# Autodesk Inventor assembly: rackpinion.ipt
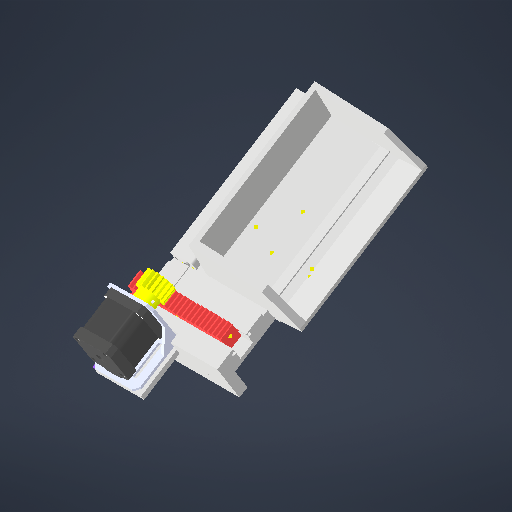
[picture p0: Inventor's stored thumbnail of the model, 512x512]
Saved by Autodesk Inventor 2027 (Build 310192000, 192)
## iProperties
Created: 2026-07-10
Part Number: rackpinion.ipt
Document SubType Name: Assembly
Designer: uchiha
Author: uchiha
## Documents named in this file (8)
- C:\Users\uchiha\Desktop\New folder\designdj\rackpinion.ipt.iam
- C:\Users\uchiha\Desktop\New folder\designdj\offloadbase.ipt
- C:\Users\uchiha\Desktop\New folder\designdj\gearsassembly.iam
- C:\Users\uchiha\Desktop\New folder\designdj\nema17-4-4kgcm-stepper-motor-1.snapshot.1\Nema17 4.4Kgcm Stepper Motor\Nema17 4.4Kgcm Stepper Motor\Nema17 4.4Kgcm Stepper Motor.iam
- C:\Users\uchiha\Desktop\New folder\designdj\Assemblyplates.iam
- C:\Users\uchiha\Documents\Inventor\Content Center Files\R2027\en-US\AS 1110\AS 1110 - M2 x 16.ipt
- C:\Users\uchiha\Documents\Inventor\Content Center Files\R2027\en-US\AS 1112 (2)\AS 1112 - M2  Type 5.ipt
- C:\Users\uchiha\Desktop\New folder\designdj\rockerconnector.ipt
## Components (9 placed, 7 different names)
1. offloadbase:1 — Mate:1, Mate:2, Mate:12, Mate:16, Mate:17
2. gearsassembly:1 [sub-assembly] — Mate:1, Mate:2, Mate:15, Mate:18, Mate:19
3. Nema17 4.4Kgcm Stepper Motor:1 [sub-assembly] — Mate:15
4. Assemblyplates:1 [sub-assembly] — Insert:1, Insert:2, Mate:7, Mate:9, Mate:10, Mate:12, Mate:16, Mate:17
5. AS 1110 - Metric M2 x 16:1 — Insert:1, Mate:5, Mate:10, Mate:13, Mate:14
6. AS 1110 - Metric M2 x 16:2 — Insert:2, Mate:6, Mate:9
7. AS 1112 (2) - Metric M2  Type 5:1 — Mate:5, Mate:13, Mate:14
8. AS 1112 (2) - Metric M2  Type 5:2 — Mate:6, Mate:7
9. rockerconnector:1 — Mate:18, Mate:19
## Relationships (17: Mate 15, Insert 2)
- Mate:1: offloadbase:1 ↔ gearsassembly:1
- Mate:2: offloadbase:1 ↔ gearsassembly:1
- Insert:1: Assemblyplates:1 ↔ AS 1110 - Metric M2 x 16:1
- Insert:2: Assemblyplates:1 ↔ AS 1110 - Metric M2 x 16:2
- Mate:5: AS 1110 - Metric M2 x 16:1 ↔ AS 1112 (2) - Metric M2  Type 5:1
- Mate:6: AS 1110 - Metric M2 x 16:2 ↔ AS 1112 (2) - Metric M2  Type 5:2
- Mate:7: Assemblyplates:1 ↔ AS 1112 (2) - Metric M2  Type 5:2
- Mate:9: Assemblyplates:1 ↔ AS 1110 - Metric M2 x 16:2
- Mate:10: Assemblyplates:1 ↔ AS 1110 - Metric M2 x 16:1
- Mate:12: offloadbase:1 ↔ Assemblyplates:1
- Mate:13: AS 1110 - Metric M2 x 16:1 ↔ AS 1112 (2) - Metric M2  Type 5:1
- Mate:14: AS 1110 - Metric M2 x 16:1 ↔ AS 1112 (2) - Metric M2  Type 5:1
- Mate:15: gearsassembly:1 ↔ Nema17 4.4Kgcm Stepper Motor:1
- Mate:16: offloadbase:1 ↔ Assemblyplates:1
- Mate:17: offloadbase:1 ↔ Assemblyplates:1
- Mate:18: gearsassembly:1 ↔ rockerconnector:1
- Mate:19: gearsassembly:1 ↔ rockerconnector:1
